# Autodesk Inventor assembly: XY Assembly
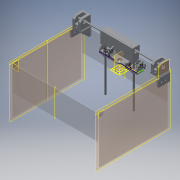
[picture p0: Inventor's stored thumbnail of the model, 180x180]
Saved by Autodesk Inventor 2016 (Build 200138000, 138)
## iProperties
Created: 2014-11-15
Part Number: XY Assembly
Document SubType Name: Assembly
Designer: Scott
Author: Scott
## Documents named in this file (12)
- C:\Users\Scott\Google Drive\Engineering Ideas and Designs\3D printer\PISCES\Parts\V5\XY Assembly.iam
- C:\Users\Scott\Google Drive\Engineering Ideas and Designs\3D printer\PISCES\Parts\V5\Front.ipt plate.ipt
- C:\Users\Scott\Google Drive\Engineering Ideas and Designs\3D printer\PISCES\Parts\V5\Side Panel.ipt
- C:\Users\Scott\Google Drive\Engineering Ideas and Designs\3D printer\PISCES\Parts\V5\Side Panelopposite.ipt
- C:\Users\Scott\Google Drive\Engineering Ideas and Designs\3D printer\PISCES\Parts\V5\Front.ipt plateopposite.ipt
- C:\Users\Scott\Google Drive\Engineering Ideas and Designs\3D printer\PISCES\Parts\V5\Ystartnew.ipt
- C:\Users\Scott\Google Drive\Engineering Ideas and Designs\3D printer\PISCES\Parts\V5\Ystartnewopposite.ipt
- C:\Users\Scott\Google Drive\Engineering Ideas and Designs\3D printer\PISCES\Parts\V5\Spinner Rail.ipt
- C:\Users\Scott\Google Drive\Engineering Ideas and Designs\3D printer\PISCES\Parts\V5\Backstop.ipt
- C:\Users\Scott\Google Drive\Engineering Ideas and Designs\3D printer\PISCES\Parts\V5\Plate Endstop and securer.ipt
- C:\Users\Scott\Google Drive\Engineering Ideas and Designs\3D printer\PISCES\Parts\V5\ZRails.ipt
- C:\Users\Scott\Google Drive\Engineering Ideas and Designs\3D printer\PISCES\Parts\V5\Crossmount.ipt
## Components (11 placed, 11 different names)
1. Front.ipt plate:1 — Mate:1, Mate:2, Mate:3
2. Side Panel:1 — Mate:4, Mate:5, Mate:6, Flush:1, Flush:2, Flush:3
3. Side Panelopposite:1
4. Front.ipt plateopposite:1 — Mate:7, Mate:8, Mate:9, Flush:6, Mate:10
5. Ystartnew:1 — Flush:1, Flush:2, Flush:3
6. Ystartnewopposite:1 — Flush:4, Flush:5
7. Spinner Rail:1 — Flush:4, Flush:5
8. Backstop:1 — Flush:6
9. Plate Endstop and securer:1 — Mate:10, Flush:7, Flush:8
10. ZRails:1 — Flush:7, Flush:8, Flush:9
11. Crossmount:1 — Flush:9
## Relationships (19: Mate 10, Flush 9)
- Mate:1: Front.ipt plate:1
- Mate:2: Front.ipt plate:1
- Mate:3: Front.ipt plate:1
- Mate:4: Side Panel:1
- Mate:5: Side Panel:1
- Mate:6: Side Panel:1
- Mate:7: Front.ipt plateopposite:1
- Mate:8: Front.ipt plateopposite:1
- Mate:9: Front.ipt plateopposite:1
- Flush:1: Side Panel:1 ↔ Ystartnew:1
- Flush:2: Side Panel:1 ↔ Ystartnew:1
- Flush:3: Side Panel:1 ↔ Ystartnew:1
- Flush:4: Ystartnewopposite:1 ↔ Spinner Rail:1
- Flush:5: Ystartnewopposite:1 ↔ Spinner Rail:1
- Flush:6: Front.ipt plateopposite:1 ↔ Backstop:1
- Mate:10: Front.ipt plateopposite:1 ↔ Plate Endstop and securer:1
- Flush:7: Plate Endstop and securer:1 ↔ ZRails:1
- Flush:8: Plate Endstop and securer:1 ↔ ZRails:1
- Flush:9: ZRails:1 ↔ Crossmount:1
